# Autodesk Inventor assembly: wheel sub assembly
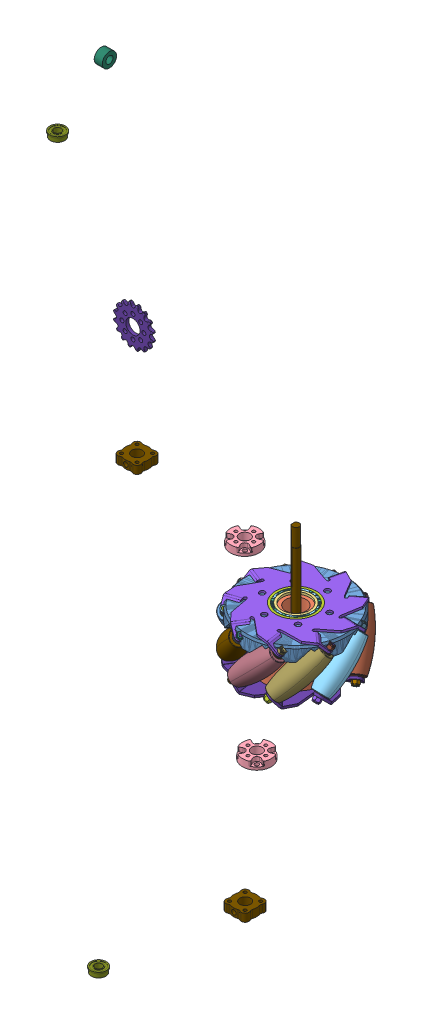
[picture p0: shaded view drawn from the shape stored in the file]
Saved by Autodesk Inventor 2017 (Build 210142000, 142)
## iProperties
Created: 2017-07-29
Part Number: wheel sub assembly
Document SubType Name: Assembly
Designer: User
Author: User
## Documents named in this file (8)
- C:\Robotics\CAD\2016-17_CAD\DriveTrain\wheel sub assembly.iam
- C:\Robotics\CAD\COTSParts\Actobotics\634 parts\634080.ipt
- C:\Robotics\CAD\COTSParts\Actobotics\545 parts\545456.ipt
- C:\Robotics\CAD\COTSParts\Actobotics\545 parts\545556.ipt
- C:\Robotics\CAD\COTSParts\Actobotics\615 parts\615102.ipt
- C:\Robotics\CAD\COTSParts\Actobotics\535 parts\535198.ipt
- C:\Robotics\CAD\COTSParts\Wheels\AndyMark Mecanum Wheels\100mm Aluminum Mecanum wheels.ipt
- C:\Robotics\CAD\COTSParts\Actobotics\collar.ipt
## Components (10 placed, 7 different names)
1. 634080:1 — Mate:1
2. 545456:1
3. 545556:1
4. 545556:2
5. 545456:2
6. 615102:1
7. 535198:1
8. 535198:2
9. 100mm Aluminum Mecanum wheels:1 — Mate:1
10. collar:1
## Relationships (1: Mate 1)
- Mate:1: 634080:1 ↔ 100mm Aluminum Mecanum wheels:1
